# Autodesk Inventor assembly: 17-0028-0076
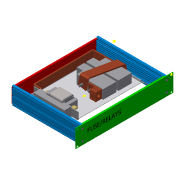
[picture p0: Inventor's stored thumbnail of the model, 180x180]
Saved by Autodesk Inventor 2016 SP2 (Build 200236200, 236)
## iProperties
Company: Universiteit van Amsterdam
Category: -
Created: 2017-03-29
Part Number: 17-0028-0076
Description: Fuse/relay box
Document SubType Name: Assembly
Designer: Daan Giesen
Authority: Reichsöllner, Lukas
Project: Digital PID Loop
Cost Center: 17-0028
User Status: Work in Progress
Preprocessor: Spatial InterOp 3D
Title: Digital PID Loop
Author: TraceParts
Revision Number: A
## Documents named in this file (13)
- D:\VaultLocalWorkingFolder\UvA_MT\Projects\2017\17-0028 Digital PID Loop\10_Assemblies\17-0028-0076.iam
- D:\VaultLocalWorkingFolder\UvA_MT\Projects\2017\17-0028 Digital PID Loop\20_3D-Models\17-0028-0047.ipt
- D:\VaultLocalWorkingFolder\UvA_MT\Projects\2017\17-0028 Digital PID Loop\20_3D-Models\17-0028-0048.ipt
- D:\VaultLocalWorkingFolder\UvA_MT\Projects\2017\17-0028 Digital PID Loop\20_3D-Models\17-0028-0050.ipt
- D:\VaultLocalWorkingFolder\UvA_MT\Projects\2017\17-0028 Digital PID Loop\20_3D-Models\17-0028-0078.ipt
- D:\VaultLocalWorkingFolder\UvA_MT\Projects\2017\17-0028 Digital PID Loop\20_3D-Models\17-0028-0086.iam
- D:\VaultLocalWorkingFolder\UvA_MT\Projects\2017\17-0028 Digital PID Loop\20_3D-Models\26388.ipt
- D:\VaultLocalWorkingFolder\UvA_MT\Projects\2017\17-0028 Digital PID Loop\20_3D-Models\17-0028-0082.ipt
- D:\VaultLocalWorkingFolder\UvA_MT\Projects\2017\17-0028 Digital PID Loop\20_3D-Models\17-0028-0085.ipt
- D:\VaultLocalWorkingFolder\UvA_MT\Projects\2017\17-0028 Digital PID Loop\20_3D-Models\17-0028-0119.ipt
- D:\VaultLocalWorkingFolder\UvA_MT\Projects\2017\17-0028 Digital PID Loop\20_3D-Models\17-0028-0120.ipt
- D:\VaultLocalWorkingFolder\UvA_MT\Projects\2017\17-0028 Digital PID Loop\20_3D-Models\17-0028-0109.ipt
- D:\VaultLocalWorkingFolder\UvA_MT\Projects\2017\17-0028 Digital PID Loop\20_3D-Models\17-0028-0110.ipt
## Components (13 placed, 12 different names)
1. 20860212_1 — Mate:1, Mate:2
2. 20860212_3
3. 20860212_5
4. 20860212_6 — Mate:7
5. 17-0028-0086:1 [sub-assembly] — Mate:1, Mate:2, Mate:4, Mate:5, Mate:7, Mate:8, Mate:13, Flush:4
6. 26388:1 — Mate:9, Mate:10, Mate:11
7. 17-0028-0082:1 — Mate:4, Mate:6, Flush:1, Flush:5, Mate:16, Mate:17, Mate:19, Mate:20, Angle:1
8. 17-0028-0082:2 — Mate:5, Mate:6, Flush:1, Mate:18
9. 17-0028-0085:1 — Mate:8, Mate:9, Mate:10, Mate:11, Mate:13, Mate:14, Flush:3, Mate:15, Flush:4, Flush:5
10. 17-0028-0119:1 — Mate:14, Flush:3, Mate:15, Mate:18
11. 17-0028-0120:1 — Mate:16, Mate:17
12. 17-0028-0109:1 — Mate:19, Mate:20, Angle:1, Mate:21, Flush:6, Flush:7
13. 17-0028-0110:1 — Mate:21, Flush:6, Flush:7
## Relationships (26: Mate 19, Flush 6, Angle 1)
- Mate:1: 20860212_1 ↔ 17-0028-0086:1
- Mate:2: 20860212_1 ↔ 17-0028-0086:1
- Mate:4 (20 mm): 17-0028-0086:1 ↔ 17-0028-0082:1
- Mate:5 (20 mm): 17-0028-0086:1 ↔ 17-0028-0082:2
- Mate:6 (10 mm): 17-0028-0082:1 ↔ 17-0028-0082:2
- Flush:1: 17-0028-0082:1 ↔ 17-0028-0082:2
- Mate:7 (10 mm): 20860212_6 ↔ 17-0028-0086:1
- Mate:8 (20 mm): 17-0028-0086:1 ↔ 17-0028-0085:1
- Mate:9: 26388:1 ↔ 17-0028-0085:1
- Mate:10: 26388:1 ↔ 17-0028-0085:1
- Mate:11 (5 mm): 26388:1 ↔ 17-0028-0085:1
- Mate:13 (20 mm): 17-0028-0086:1 ↔ 17-0028-0085:1
- Mate:14: 17-0028-0085:1 ↔ 17-0028-0119:1
- Flush:3 (-4 mm): 17-0028-0085:1 ↔ 17-0028-0119:1
- Mate:15: 17-0028-0085:1 ↔ 17-0028-0119:1
- Flush:4: 17-0028-0086:1 ↔ 17-0028-0085:1
- Flush:5: 17-0028-0082:1 ↔ 17-0028-0085:1
- Mate:16 (10 mm): 17-0028-0082:1 ↔ 17-0028-0120:1
- Mate:17: 17-0028-0082:1 ↔ 17-0028-0120:1
- Mate:18: 17-0028-0082:2 ↔ 17-0028-0119:1
- Mate:19: 17-0028-0082:1 ↔ 17-0028-0109:1
- Mate:20: 17-0028-0082:1 ↔ 17-0028-0109:1
- Angle:1 (0 deg): 17-0028-0082:1 ↔ 17-0028-0109:1
- Mate:21: 17-0028-0109:1 ↔ 17-0028-0110:1
- Flush:6: 17-0028-0109:1 ↔ 17-0028-0110:1
- Flush:7: 17-0028-0109:1 ↔ 17-0028-0110:1
